# Autodesk Inventor assembly: Pickle Floorplan with straps not wood
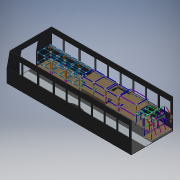
[picture p0: Inventor's stored thumbnail of the model, 180x180]
Saved by Autodesk Inventor 2018.2 (Build 222227000, 227)
## iProperties
Created: 2018-02-27
Part Number: Pickle Floorplan with straps not wood
Document SubType Name: Assembly
Designer: owner
Author: owner
## Documents named in this file (11)
- Z:\The Pickle - 4 - Copy\Final Carts\Pickle Floorplan.iam
- Z:\The Pickle - 4 - Copy\Final Carts\Pickle Interior Assembly\Pickle Interior.ipt
- Z:\The Pickle - 4 - Copy\Final Carts\Mellie Cart\Mellie Cart.iam
- Z:\The Pickle - 4 - Copy\Final Carts\T-Bone Cart\T-Bone Cart.iam
- Z:\The Pickle - 4 - Copy\Final Carts\Sax Cart\Bari Sax Cart.iam
- Z:\The Pickle - 4 - Copy\Final Carts\Sax Cart\Tenor Sax Cart.iam
- Z:\The Pickle - 4 - Copy\Final Carts\Euph Cart\Euph Cart.iam
- Z:\The Pickle - 4 - Copy\Final Carts\Mellie Cart\Mellie Side Cart.iam
- Z:\The Pickle - 4 - Copy\Final Carts\Locking Mech\Snap Track 10ft.ipt
- Z:\The Pickle - 4 - Copy\Final Carts\Locking Mech\Snap Track Single Snap.ipt
- Z:\The Pickle - 4 - Copy\Final Carts\Locking Mech\Snap Track Ring.ipt
## Components (29 placed, 10 different names)
1. Pickle Interior:1 — Mate:2, Mate:3, Mate:4, Mate:7, Mate:8, Tangent:1, Mate:10, Tangent:3, Tangent:4, Tangent:5, Mate:13, Mate:14, Mate:15, Tangent:6, Tangent:7, Tangent:8, Tangent:9, Tangent:10, Tangent:11, Mate:82, Mate:83, Mate:84, Mate:86, Mate:87, Mate:89
2. Snap Track 10ft:3 — Mate:84, Flush:32, Mate:85, Flush:44
3. Snap Track Single Snap:1 — Flush:18, Flush:42
4. Snap Track Single Snap:2 — Flush:19, Mate:82, Flush:43
5. Snap Track Single Snap:3 — Flush:18, Flush:19, Flush:42
6. Snap Track Single Snap:4 — Mate:86, Flush:43, Flush:44
7. Snap Track Ring:1 — Flush:29, Flush:30, Flush:33, Flush:34, Flush:35
8. Snap Track Ring:2 — Flush:28, Flush:29, Flush:35, Flush:36
9. Snap Track Ring:3 — Flush:27, Flush:28, Flush:36, Flush:37
10. Snap Track Ring:4 — Flush:30, Flush:34
11. Snap Track Ring:5 — Flush:26, Flush:27, Flush:37, Flush:38
12. Snap Track Ring:6 — Flush:22, Flush:25, Flush:38, Flush:39
13. Snap Track Ring:7 — Flush:31
14. Snap Track Ring:8 — Flush:24, Flush:25, Mate:83
15. Snap Track Ring:9 — Flush:23, Flush:24
16. Snap Track Ring:10 — Flush:23, Flush:31
17. Snap Track Ring:11 — Flush:22, Flush:26, Flush:39
18. Snap Track 10ft:1 — Flush:32, Mate:85, Flush:33
19. Snap Track 10ft:5 — Flush:40, Flush:41, Mate:87, Mate:88
20. Snap Track 10ft:6 — Flush:40, Flush:41, Mate:88
21. Snap Track Single Snap:5 — Mate:89
22. Tenor Sax Cart:1 [sub-assembly] — Mate:8, Tangent:10, Tangent:11
23. Euph Cart:1 [sub-assembly] — Mate:14, Tangent:8, Tangent:9
24. Mellie Side Cart:1 [sub-assembly] — Mate:15, Tangent:6, Tangent:7
25. T-Bone Cart:3 [sub-assembly] — Mate:2, Flush:1, Flush:2
26. T-Bone Cart:1 [sub-assembly] — Mate:4, Flush:1, Tangent:4, Tangent:5
27. T-Bone Cart:2 [sub-assembly] — Mate:3, Flush:2
28. Bari Sax Cart:1 [sub-assembly] — Mate:7, Tangent:1, Tangent:3
29. Mellie Cart:1 [sub-assembly] — Mate:10, Mate:13
## Relationships (54: Flush 27, Mate 17, Tangent 10)
- Mate:2 (120.65 mm): Pickle Interior:1 ↔ T-Bone Cart:3
- Mate:3 (120.65 mm): Pickle Interior:1 ↔ T-Bone Cart:2
- Mate:4 (120.65 mm): Pickle Interior:1 ↔ T-Bone Cart:1
- Mate:7 (73.025 mm): Pickle Interior:1 ↔ Bari Sax Cart:1
- Mate:8 (120.65 mm): Pickle Interior:1 ↔ Tenor Sax Cart:1
- Tangent:1: Pickle Interior:1 ↔ Bari Sax Cart:1
- Flush:1: T-Bone Cart:3 ↔ T-Bone Cart:1
- Flush:2: T-Bone Cart:3 ↔ T-Bone Cart:2
- Mate:10: Pickle Interior:1 ↔ Mellie Cart:1
- Tangent:3: Pickle Interior:1 ↔ Bari Sax Cart:1
- Tangent:4: Pickle Interior:1 ↔ T-Bone Cart:1
- Tangent:5: Pickle Interior:1 ↔ T-Bone Cart:1
- Mate:13 (247.65 mm): Pickle Interior:1 ↔ Mellie Cart:1
- Mate:14 (120.65 mm): Pickle Interior:1 ↔ Euph Cart:1
- Mate:15 (120.65 mm): Pickle Interior:1 ↔ Mellie Side Cart:1
- Tangent:6 (17.907 mm): Pickle Interior:1 ↔ Mellie Side Cart:1
- Tangent:7 (17.907 mm): Pickle Interior:1 ↔ Mellie Side Cart:1
- Tangent:8 (17.907 mm): Pickle Interior:1 ↔ Euph Cart:1
- Tangent:9 (17.907 mm): Pickle Interior:1 ↔ Euph Cart:1
- Tangent:10 (5.0546 mm): Pickle Interior:1 ↔ Tenor Sax Cart:1
- Tangent:11 (5.0546 mm): Pickle Interior:1 ↔ Tenor Sax Cart:1
- Flush:18: Snap Track Single Snap:1 ↔ Snap Track Single Snap:3
- Flush:19: Snap Track Single Snap:2 ↔ Snap Track Single Snap:3
- Mate:82: Pickle Interior:1 ↔ Snap Track Single Snap:2
- Flush:22: Snap Track Ring:6 ↔ Snap Track Ring:11
- Flush:23: Snap Track Ring:9 ↔ Snap Track Ring:10
- Flush:24: Snap Track Ring:8 ↔ Snap Track Ring:9
- Flush:25: Snap Track Ring:6 ↔ Snap Track Ring:8
- Flush:26: Snap Track Ring:5 ↔ Snap Track Ring:11
- Flush:27: Snap Track Ring:3 ↔ Snap Track Ring:5
- Flush:28: Snap Track Ring:2 ↔ Snap Track Ring:3
- Flush:29: Snap Track Ring:1 ↔ Snap Track Ring:2
- Flush:30: Snap Track Ring:1 ↔ Snap Track Ring:4
- Flush:31: Snap Track Ring:7 ↔ Snap Track Ring:10
- Mate:83: Pickle Interior:1 ↔ Snap Track Ring:8
- Mate:84: Pickle Interior:1 ↔ Snap Track 10ft:3
- Flush:32: Snap Track 10ft:3 ↔ Snap Track 10ft:1
- Mate:85: Snap Track 10ft:3 ↔ Snap Track 10ft:1
- Mate:86: Pickle Interior:1 ↔ Snap Track Single Snap:4
- Flush:33: Snap Track Ring:1 ↔ Snap Track 10ft:1
- Flush:34: Snap Track Ring:1 ↔ Snap Track Ring:4
- Flush:35: Snap Track Ring:1 ↔ Snap Track Ring:2
- Flush:36: Snap Track Ring:2 ↔ Snap Track Ring:3
- Flush:37: Snap Track Ring:3 ↔ Snap Track Ring:5
- Flush:38: Snap Track Ring:5 ↔ Snap Track Ring:6
- Flush:39: Snap Track Ring:6 ↔ Snap Track Ring:11
- Flush:40: Snap Track 10ft:5 ↔ Snap Track 10ft:6
- Flush:41: Snap Track 10ft:5 ↔ Snap Track 10ft:6
- Mate:87: Pickle Interior:1 ↔ Snap Track 10ft:5
- Mate:88: Snap Track 10ft:5 ↔ Snap Track 10ft:6
- Mate:89: Pickle Interior:1 ↔ Snap Track Single Snap:5
- Flush:42: Snap Track Single Snap:1 ↔ Snap Track Single Snap:3
- Flush:43: Snap Track Single Snap:2 ↔ Snap Track Single Snap:4
- Flush:44: Snap Track 10ft:3 ↔ Snap Track Single Snap:4
